# Autodesk Inventor assembly: BaratronBox
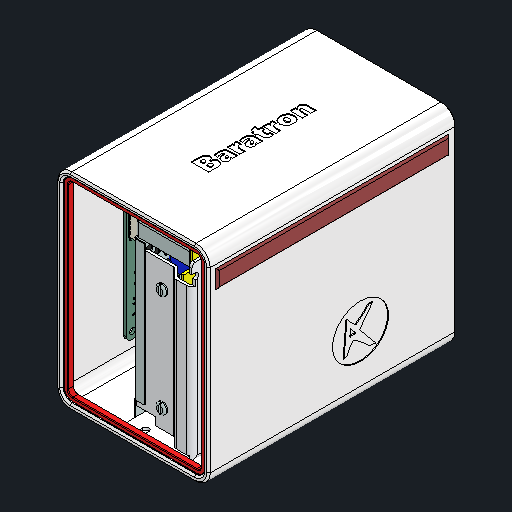
[picture p0: Inventor's stored thumbnail of the model, 512x512]
Saved by Autodesk Inventor 2026 (Build 300175050, 175E)
## iProperties
Created: 2025-12-13
Part Number: BaratronBox
Document SubType Name: Assembly
Designer: queezz
Author: queezz
## Documents named in this file (4)
- C:\Users\queezz\Dropbox\Drawings\PIHTI\ElectronicsBox\BaratronBox\BaratronBox.iam
- C:\Users\queezz\Dropbox\Drawings\PIHTI\ElectronicsBox\BaratronBox\enclosure-baratron.ipt
- C:\Users\queezz\Dropbox\Drawings\PIHTI\ContentCenter\Electrics\MEAN WELL RT-65D\MEAN WELL RT-65D.iam
- C:\Users\queezz\Dropbox\Drawings\PIHTI\ElectronicsBox\BaratronBox\TempLoggerRev1.iam
## Components (3 placed, 3 different names)
1. enclosure-baratron:1 — Mate:1, Mate:2, Mate:3
2. MEAN WELL RT-65D:1 [sub-assembly] — Mate:1, Mate:2
3. TempLoggerRev1:1 [sub-assembly] — Mate:3
## Relationships (3: Mate 3)
- Mate:1: enclosure-baratron:1 ↔ MEAN WELL RT-65D:1
- Mate:2: enclosure-baratron:1 ↔ MEAN WELL RT-65D:1
- Mate:3: enclosure-baratron:1 ↔ TempLoggerRev1:1
